# Autodesk Inventor assembly: launch system
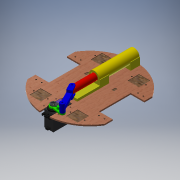
[picture p0: Inventor's stored thumbnail of the model, 180x180]
Saved by Autodesk Inventor 2017 (Build 210142000, 142)
## iProperties
Created: 2019-12-07
Part Number: launch system
Document SubType Name: Assembly
Designer: User
Author: User
## Documents named in this file (10)
- D:\台大\大三上 108-1\機械設計\launch system.iam
- D:\台大\大三上 108-1\機械設計\底盤.ipt
- D:\台大\大三上 108-1\機械設計\筷子套.ipt
- D:\台大\大三上 108-1\機械設計\筷子套軸.ipt
- D:\台大\大三上 108-1\機械設計\蓋子.ipt
- D:\台大\大三上 108-1\機械設計\蓋子2.ipt
- D:\台大\大三上 108-1\機械設計\彈簧套.ipt
- D:\台大\大三上 108-1\機械設計\轉軸.ipt
- D:\台大\大三上 108-1\機械設計\Servomotor.ipt
- D:\台大\大三上 108-1\機械設計\Servomotor-1.ipt
## Components (9 placed, 9 different names)
1. 底盤:1 — Mate:1, Mate:7, Mate:18, Mate:21
2. 筷子套:1 — Mate:8, Mate:16, Flush:5
3. 筷子套軸:1 — Mate:2, Mate:3, Mate:16, Flush:5
4. 蓋子:1 — Mate:6, Flush:2, Mate:9
5. 蓋子2:1 — Mate:1, Mate:4, Mate:5, Mate:6, Flush:2, Mate:7, Mate:8, Mate:9
6. 彈簧套:1 — Mate:4, Mate:5
7. 轉軸:1 — Mate:2, Mate:3, Mate:11, Mate:12, Mate:14, Mate:19
8. Servomotor:1 — Mate:11, Mate:14, Mate:18, Mate:21
9. Servomotor-1:1 — Mate:12, Mate:19
## Relationships (18: Mate 16, Flush 2)
- Mate:1: 底盤:1 ↔ 蓋子2:1
- Mate:2: 筷子套軸:1 ↔ 轉軸:1
- Mate:3: 筷子套軸:1 ↔ 轉軸:1
- Mate:4: 蓋子2:1 ↔ 彈簧套:1
- Mate:5: 蓋子2:1 ↔ 彈簧套:1
- Mate:6: 蓋子:1 ↔ 蓋子2:1
- Flush:2: 蓋子:1 ↔ 蓋子2:1
- Mate:7: 底盤:1 ↔ 蓋子2:1
- Mate:8: 筷子套:1 ↔ 蓋子2:1
- Mate:9: 蓋子:1 ↔ 蓋子2:1
- Mate:11: 轉軸:1 ↔ Servomotor:1
- Mate:12: 轉軸:1 ↔ Servomotor-1:1
- Mate:14: 轉軸:1 ↔ Servomotor:1
- Mate:16: 筷子套:1 ↔ 筷子套軸:1
- Flush:5: 筷子套:1 ↔ 筷子套軸:1
- Mate:18: 底盤:1 ↔ Servomotor:1
- Mate:19 (1 mm): 轉軸:1 ↔ Servomotor-1:1
- Mate:21 (1 mm): 底盤:1 ↔ Servomotor:1
